# Autodesk Inventor assembly: tr2
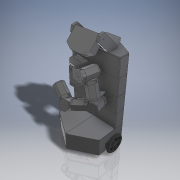
[picture p0: Inventor's stored thumbnail of the model, 180x180]
Saved by Autodesk Inventor 2017 (Build 210142000, 142)
## iProperties
Created: 2018-10-17
Part Number: tr2
Document SubType Name: Assembly
Designer: Administrator
Author: Administrator
## Documents named in this file (5)
- C:\Users\Dell\Documents\GitHub\tr2\TR2.iam
- C:\Users\Dell\Documents\GitHub\tr2\Base\Base.iam
- C:\Users\Dell\Documents\GitHub\tr2\Body\Body.iam
- C:\Users\Dell\Documents\GitHub\tr2\Arm\Arm.iam
- C:\Users\Dell\Documents\GitHub\tr2\Head\Head.iam
## Components (4 placed, 4 different names)
1. Base:1 [sub-assembly] — Mate:2, Mate:3, Mate:4, Mate:5, Mate:6, Mate:8, Mate:9, Mate:12, Flush:2
2. Body:1 [sub-assembly] — Mate:6, Mate:8, Mate:9, Mate:11, Flush:1, Mate:13
3. Arm:1 [sub-assembly] — Mate:12, Flush:2, Mate:13
4. Head:1 [sub-assembly] — Mate:11, Flush:1
## Relationships (12: Mate 10, Flush 2)
- Mate:2 (40 mm): Base:1
- Mate:3: Base:1
- Mate:4: Base:1
- Mate:5: Base:1
- Mate:6: Base:1 ↔ Body:1
- Mate:8: Base:1 ↔ Body:1
- Mate:9: Base:1 ↔ Body:1
- Mate:11: Body:1 ↔ Head:1
- Flush:1 (125 mm): Body:1 ↔ Head:1
- Mate:12: Base:1 ↔ Arm:1
- Flush:2 (206.5 mm): Base:1 ↔ Arm:1
- Mate:13: Body:1 ↔ Arm:1
